# Autodesk Inventor assembly: Ensamble Final
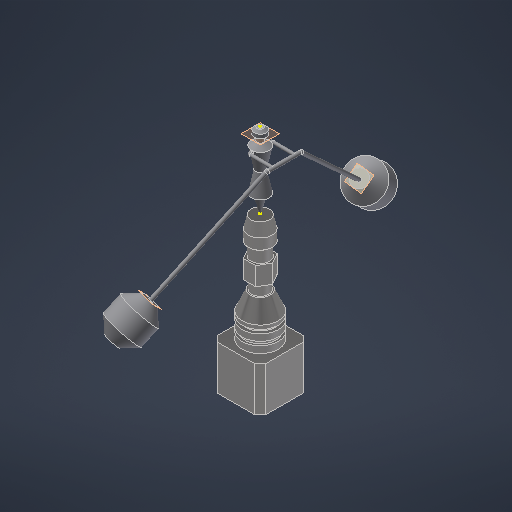
[picture p0: Inventor's stored thumbnail of the model, 512x512]
Saved by Autodesk Inventor 2026 (Build 300175000, 175)
## iProperties
Created: 2025-07-07
Part Number: Ensamble Final
Document SubType Name: Assembly
Designer: feder
Author: feder
## Documents named in this file (8)
- C:\Users\feder\OneDrive - Universidad de Antioquia\Desktop\UdeA\2025-1\Mecanizado\Bailarina\Ensamble Final.iam
- C:\Users\feder\OneDrive - Universidad de Antioquia\Desktop\UdeA\2025-1\Mecanizado\Bailarina\Base.ipt
- C:\Users\feder\OneDrive - Universidad de Antioquia\Desktop\UdeA\2025-1\Mecanizado\Bailarina\Soporte Intermedio.ipt
- C:\Users\feder\OneDrive - Universidad de Antioquia\Desktop\UdeA\2025-1\Mecanizado\Bailarina\Soporte Bailarina.ipt
- C:\Users\feder\OneDrive - Universidad de Antioquia\Desktop\UdeA\2025-1\Mecanizado\Bailarina\BAILARINA.ipt
- C:\Users\feder\OneDrive - Universidad de Antioquia\Desktop\UdeA\2025-1\Mecanizado\Bailarina\BRAZOS BAILARINA.ipt
- C:\Users\feder\OneDrive - Universidad de Antioquia\Desktop\UdeA\2025-1\Mecanizado\Bailarina\SOPORTE PESAS.ipt
- C:\Users\feder\OneDrive - Universidad de Antioquia\Desktop\UdeA\2025-1\Mecanizado\Bailarina\PESAS BAILARINA.ipt
## Components (8 placed, 7 different names)
1. Base:1 — Mate:1, Mate:2
2. Soporte Intermedio:1 — Mate:1, Mate:2, Mate:3, Mate:4
3. Soporte Bailarina:1 — Mate:3, Mate:4, Mate:5
4. BAILARINA:1 — Mate:5, Mate:6
5. BRAZOS BAILARINA:1 — Mate:6, Mate:7
6. SOPORTE PESAS:1 — Mate:7, Mate:8, Mate:9
7. PESAS BAILARINA:1 — Mate:8
8. PESAS BAILARINA:2 — Mate:9
## Relationships (9: Mate 9)
- Mate:1: Base:1 ↔ Soporte Intermedio:1
- Mate:2: Base:1 ↔ Soporte Intermedio:1
- Mate:3: Soporte Intermedio:1 ↔ Soporte Bailarina:1
- Mate:4: Soporte Intermedio:1 ↔ Soporte Bailarina:1
- Mate:5 (19.45 mm): Soporte Bailarina:1 ↔ BAILARINA:1
- Mate:6: BAILARINA:1 ↔ BRAZOS BAILARINA:1
- Mate:7: BRAZOS BAILARINA:1 ↔ SOPORTE PESAS:1
- Mate:8: SOPORTE PESAS:1 ↔ PESAS BAILARINA:1
- Mate:9: SOPORTE PESAS:1 ↔ PESAS BAILARINA:2
